# Autodesk Inventor assembly: POM_T5_02
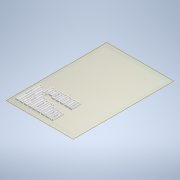
[picture p0: Inventor's stored thumbnail of the model, 180x180]
Saved by Autodesk Inventor 2020 (Build 240168000, 168)
## iProperties
Created: 2021-08-27
Part Number: POM_T5_02
Document SubType Name: Assembly
Designer: Masato
Author: Masato
## Documents named in this file (19)
- C:\Users\Masato\Documents\Inventor\CIT Brains_Inventor\OpenPlatform_ver3_0\cam\POM_T5_02.iam
- C:\Users\Masato\Documents\Inventor\CIT Brains_Inventor\OpenPlatform_ver3_0\cam\Disposable_Board.ipt
- C:\Users\Masato\Documents\Inventor\CIT Brains_Inventor\OpenPlatform_ver3_0\JIG\BackLink_diagonal_jig.ipt
- C:\Users\Masato\Documents\Inventor\CIT Brains_Inventor\OpenPlatform_ver3_0\JIG\Camera_side_frame_jig.ipt
- C:\Users\Masato\Documents\Inventor\CIT Brains_Inventor\OpenPlatform_ver3_0\JIG\Foot_root_block_jig.ipt
- C:\Users\Masato\Documents\Inventor\CIT Brains_Inventor\OpenPlatform_ver3_0\JIG\ForeArm_diagonal_jig_01.ipt
- C:\Users\Masato\Documents\Inventor\CIT Brains_Inventor\OpenPlatform_ver3_0\JIG\ForeArm_diagonal_jig_02.ipt
- C:\Users\Masato\Documents\Inventor\CIT Brains_Inventor\OpenPlatform_ver3_0\JIG\ForeArm_diagonal_jig_03.ipt
- C:\Users\Masato\Documents\Inventor\CIT Brains_Inventor\OpenPlatform_ver3_0\JIG\FrontLink_diagonal_jig.ipt
- C:\Users\Masato\Documents\Inventor\CIT Brains_Inventor\OpenPlatform_ver3_0\JIG\Head_diagonal_jig.ipt
- C:\Users\Masato\Documents\Inventor\CIT Brains_Inventor\OpenPlatform_ver3_0\JIG\Head_horn_frame_jig.ipt
- C:\Users\Masato\Documents\Inventor\CIT Brains_Inventor\OpenPlatform_ver3_0\JIG\Leg_joint_yaw_frame_jig.ipt
- C:\Users\Masato\Documents\Inventor\CIT Brains_Inventor\OpenPlatform_ver3_0\JIG\Shoulder_horn_frame_jig.ipt
- C:\Users\Masato\Documents\Inventor\CIT Brains_Inventor\OpenPlatform_ver3_0\JIG\Trunk_ampit_frame_jig_01.ipt
- C:\Users\Masato\Documents\Inventor\CIT Brains_Inventor\OpenPlatform_ver3_0\JIG\Trunk_ampit_frame_jig_02.ipt
- C:\Users\Masato\Documents\Inventor\CIT Brains_Inventor\OpenPlatform_ver3_0\JIG\Trunk_chest_back_forth_frame_jig_01.ipt
- C:\Users\Masato\Documents\Inventor\CIT Brains_Inventor\OpenPlatform_ver3_0\JIG\Trunk_chest_back_forth_frame_jig_02.ipt
- C:\Users\Masato\Documents\Inventor\CIT Brains_Inventor\OpenPlatform_ver3_0\JIG\Trunk_lower_flank_frame_jig.ipt
- C:\Users\Masato\Documents\Inventor\CIT Brains_Inventor\OpenPlatform_ver3_0\JIG\UpperArm_diagonal_jig.ipt
## Components (18 placed, 18 different names)
1. Disposable_Board:1 — メイト:2, メイト:1, フラッシュ:1, フラッシュ:2
2. BackLink_diagonal_jig:1 — メイト:4, フラッシュ:11, フラッシュ:18
3. Camera_side_frame_jig:1 — メイト:6, フラッシュ:4, メイト:21, メイト:22, フラッシュ:23, メイト:28
4. Foot_root_block_jig:1 — メイト:5, フラッシュ:13, フラッシュ:20
5. ForeArm_diagonal_jig_01:1 — メイト:8, フラッシュ:10, メイト:27, フラッシュ:17
6. ForeArm_diagonal_jig_02:1 — メイト:7, フラッシュ:15, フラッシュ:22
7. ForeArm_diagonal_jig_03:1 — メイト:9, フラッシュ:16, フラッシュ:23, メイト:28
8. FrontLink_diagonal_jig:1 — メイト:10, フラッシュ:5, メイト:22, メイト:23, フラッシュ:22
9. Head_diagonal_jig:1 — メイト:15, フラッシュ:14, フラッシュ:21
10. Head_horn_frame_jig:1 — メイト:16, フラッシュ:12, フラッシュ:19
11. Leg_joint_yaw_frame_jig:1 — メイト:19, フラッシュ:11, フラッシュ:12, フラッシュ:13, フラッシュ:14, フラッシュ:15, フラッシュ:16, フラッシュ:17
12. Shoulder_horn_frame_jig:1 — メイト:11, フラッシュ:9, メイト:26, メイト:27, フラッシュ:18
13. Trunk_ampit_frame_jig_01:1 — メイト:17, フラッシュ:6, メイト:23, メイト:24, フラッシュ:21
14. Trunk_ampit_frame_jig_02:1 — メイト:18, フラッシュ:7, メイト:24, メイト:25, フラッシュ:20
15. Trunk_chest_back_forth_frame_jig_01:1 — メイト:14, フラッシュ:3, フラッシュ:4, フラッシュ:5, フラッシュ:6, フラッシュ:7, フラッシュ:8, フラッシュ:9, フラッシュ:10, メイト:20
16. Trunk_chest_back_forth_frame_jig_02:1 — メイト:12, フラッシュ:8, メイト:25, メイト:26, フラッシュ:19
17. Trunk_lower_flank_frame_jig:1 — メイト:13, フラッシュ:3, メイト:20, メイト:21
18. UpperArm_diagonal_jig:1
## Relationships (50: Mate 27, Flush 23)
- メイト:2 [Mate]: Disposable_Board:1
- メイト:1 [Mate]: Disposable_Board:1
- フラッシュ:1 [Flush]: Disposable_Board:1
- フラッシュ:2 [Flush]: Disposable_Board:1
- メイト:4 [Mate]: BackLink_diagonal_jig:1
- メイト:5 [Mate]: Foot_root_block_jig:1
- メイト:6 [Mate]: Camera_side_frame_jig:1
- メイト:7 [Mate]: ForeArm_diagonal_jig_02:1
- メイト:8 [Mate]: ForeArm_diagonal_jig_01:1
- メイト:9 [Mate]: ForeArm_diagonal_jig_03:1
- メイト:10 [Mate]: FrontLink_diagonal_jig:1
- メイト:11 [Mate]: Shoulder_horn_frame_jig:1
- メイト:12 [Mate]: Trunk_chest_back_forth_frame_jig_02:1
- メイト:13 [Mate]: Trunk_lower_flank_frame_jig:1
- メイト:14 [Mate]: Trunk_chest_back_forth_frame_jig_01:1
- メイト:15 [Mate]: Head_diagonal_jig:1
- メイト:16 [Mate]: Head_horn_frame_jig:1
- メイト:17 [Mate]: Trunk_ampit_frame_jig_01:1
- メイト:18 [Mate]: Trunk_ampit_frame_jig_02:1
- メイト:19 [Mate]: Leg_joint_yaw_frame_jig:1
- フラッシュ:3 [Flush]: Trunk_chest_back_forth_frame_jig_01:1 ↔ Trunk_lower_flank_frame_jig:1
- フラッシュ:4 [Flush]: Camera_side_frame_jig:1 ↔ Trunk_chest_back_forth_frame_jig_01:1
- フラッシュ:5 [Flush]: FrontLink_diagonal_jig:1 ↔ Trunk_chest_back_forth_frame_jig_01:1
- フラッシュ:6 [Flush]: Trunk_ampit_frame_jig_01:1 ↔ Trunk_chest_back_forth_frame_jig_01:1
- フラッシュ:7 [Flush]: Trunk_ampit_frame_jig_02:1 ↔ Trunk_chest_back_forth_frame_jig_01:1
- フラッシュ:8 [Flush]: Trunk_chest_back_forth_frame_jig_01:1 ↔ Trunk_chest_back_forth_frame_jig_02:1
- フラッシュ:9 [Flush]: Shoulder_horn_frame_jig:1 ↔ Trunk_chest_back_forth_frame_jig_01:1
- フラッシュ:10 [Flush]: ForeArm_diagonal_jig_01:1 ↔ Trunk_chest_back_forth_frame_jig_01:1
- フラッシュ:11 [Flush]: BackLink_diagonal_jig:1 ↔ Leg_joint_yaw_frame_jig:1
- フラッシュ:12 [Flush]: Head_horn_frame_jig:1 ↔ Leg_joint_yaw_frame_jig:1
- フラッシュ:13 [Flush]: Foot_root_block_jig:1 ↔ Leg_joint_yaw_frame_jig:1
- フラッシュ:14 [Flush]: Head_diagonal_jig:1 ↔ Leg_joint_yaw_frame_jig:1
- フラッシュ:15 [Flush]: ForeArm_diagonal_jig_02:1 ↔ Leg_joint_yaw_frame_jig:1
- フラッシュ:16 [Flush]: ForeArm_diagonal_jig_03:1 ↔ Leg_joint_yaw_frame_jig:1
- メイト:20 [Mate] (3 mm): Trunk_chest_back_forth_frame_jig_01:1 ↔ Trunk_lower_flank_frame_jig:1
- メイト:21 [Mate] (3 mm): Camera_side_frame_jig:1 ↔ Trunk_lower_flank_frame_jig:1
- メイト:22 [Mate] (3 mm): Camera_side_frame_jig:1 ↔ FrontLink_diagonal_jig:1
- メイト:23 [Mate] (3 mm): FrontLink_diagonal_jig:1 ↔ Trunk_ampit_frame_jig_01:1
- メイト:24 [Mate] (3 mm): Trunk_ampit_frame_jig_01:1 ↔ Trunk_ampit_frame_jig_02:1
- メイト:25 [Mate] (3 mm): Trunk_ampit_frame_jig_02:1 ↔ Trunk_chest_back_forth_frame_jig_02:1
- メイト:26 [Mate] (3 mm): Shoulder_horn_frame_jig:1 ↔ Trunk_chest_back_forth_frame_jig_02:1
- メイト:27 [Mate] (3 mm): ForeArm_diagonal_jig_01:1 ↔ Shoulder_horn_frame_jig:1
- フラッシュ:17 [Flush]: ForeArm_diagonal_jig_01:1 ↔ Leg_joint_yaw_frame_jig:1
- フラッシュ:18 [Flush]: BackLink_diagonal_jig:1 ↔ Shoulder_horn_frame_jig:1
- フラッシュ:19 [Flush]: Head_horn_frame_jig:1 ↔ Trunk_chest_back_forth_frame_jig_02:1
- フラッシュ:20 [Flush]: Foot_root_block_jig:1 ↔ Trunk_ampit_frame_jig_02:1
- フラッシュ:21 [Flush]: Head_diagonal_jig:1 ↔ Trunk_ampit_frame_jig_01:1
- フラッシュ:22 [Flush]: ForeArm_diagonal_jig_02:1 ↔ FrontLink_diagonal_jig:1
- フラッシュ:23 [Flush]: Camera_side_frame_jig:1 ↔ ForeArm_diagonal_jig_03:1
- メイト:28 [Mate] (3 mm): Camera_side_frame_jig:1 ↔ ForeArm_diagonal_jig_03:1
